# Autodesk Inventor assembly: VersaPlanetary_v2_2 Stage_10_1_with_NEO 550_90 deg drive
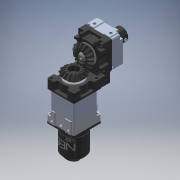
[picture p0: Inventor's stored thumbnail of the model, 180x180]
Saved by Autodesk Inventor 2018.3 (Build 223284000, 284)
## iProperties
Created: 2018-09-07
Part Number: VersaPlanetary_v2_2 Stage_10_1_with_NEO 550_90 deg drive
Description: STEP AP214
Document SubType Name: Assembly
Designer: carls
Sending System: SolidWorks 2017
Preprocessor: SwSTEP 2.0
Title: VP Input to 2X Ring Gears to 90 Degree to VP Output.STEP
Revision Number: ANY
## Documents named in this file (13)
- C:\Users\carls\Documents\GrabCAD\Infinite Recharge 2020\Build season\VersaPlanetary_v2_2 Stage_10_1_with_NEO 550_90 deg drive.iam
- C:\Users\carls\Downloads\217-6293-000 Rev1.iam
- C:\Users\carls\Downloads\VersaPlanetary Input Blocks_VP Input Block.iam
- C:\Users\carls\Downloads\VersaPlanetary Output Blocks_VP Output Block.iam
- C:\Users\carls\Downloads\VersaPlanetary Ring Gears_VP Ring Gear.iam
- C:\Users\carls\Documents\GrabCAD\Infinite Recharge 2020\Build season\217-2816-001 Rev1.ipt
- C:\Users\carls\Downloads\VersaPlanetary Gear Sets_10_1 (217-2820).iam
- C:\Users\carls\Downloads\217-2820-000 Rev2_Public.iam
- C:\Users\carls\Downloads\#8-32 SHCS, Grade 8 Steel Rev2_SSA0832-2250ZB.ipt
- C:\Users\carls\Downloads\#8-32 SHCS, Grade 8 Steel Rev2_SSA0832-0875ZB.ipt
- C:\Users\carls\Documents\GrabCAD\Infinite Recharge 2020\Build season\Universal_Female_Output_Shaft_1_2_Hex_.iam
- C:\Users\carls\Documents\GrabCAD\Infinite Recharge 2020\Build season\217-2822-001 Rev4.ipt
- C:\Users\carls\Documents\GrabCAD\Infinite Recharge 2020\Build season\REV Neo 550.ipt
## Components (14 placed, 14 different names)
1. 217-6293-000 Rev1_1 [sub-assembly]
2. VersaPlanetary Input Blocks_VP Input Block_2 [sub-assembly] — Insert:2, Angle:1, Insert:3
3. VersaPlanetary Output Blocks_VP Output Block_3 [sub-assembly] — Insert:1
4. VersaPlanetary Ring Gears_VP Ring Gear_5 [sub-assembly]
5. 217-2816-001 Rev1_6 — Insert:3
6. VersaPlanetary Gear Sets_10:1 (217-2820)_7 [sub-assembly]
7. 217-2820-000 Rev2_Public_8 [sub-assembly]
8. #8-32 SHCS, Grade 8 Steel Rev2_SSA0832-2250ZB_9
9. #8-32 SHCS, Grade 8 Steel Rev2_SSA0832-0875ZB_10
10. #8-32 SHCS, Grade 8 Steel Rev2_SSA0832-0875ZB_11
11. #8-32 SHCS, Grade 8 Steel Rev2_SSA0832-2250ZB_12
12. Universal_Female_Output_Shaft_1_2_Hex_:1 [sub-assembly] — Insert:1
13. 217-2822-001 Rev4:1 — Insert:2, Angle:1, Insert:4
14. REV Neo 550:1 — Insert:4
## Relationships (5: Insert 4, Angle 1)
- Insert:1: VersaPlanetary Output Blocks_VP Output Block_3 ↔ Universal_Female_Output_Shaft_1_2_Hex_:1
- Insert:2: VersaPlanetary Input Blocks_VP Input Block_2 ↔ 217-2822-001 Rev4:1
- Angle:1 (0 deg): VersaPlanetary Input Blocks_VP Input Block_2 ↔ 217-2822-001 Rev4:1
- Insert:3: VersaPlanetary Input Blocks_VP Input Block_2 ↔ 217-2816-001 Rev1_6
- Insert:4: 217-2822-001 Rev4:1 ↔ REV Neo 550:1
